# Autodesk Inventor assembly: Assembly1
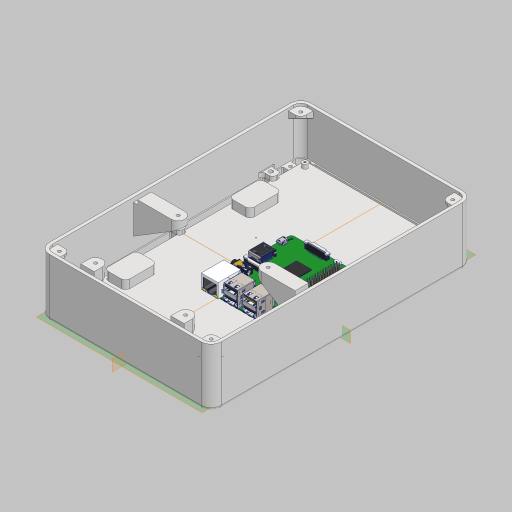
[picture p0: Inventor's stored thumbnail of the model, 512x512]
Saved by Autodesk Inventor 2024 (Build 280153000, 153)
## iProperties
Created: 2024-11-22
Part Number: Assembly1
Document SubType Name: Assembly
Designer: Stefano
Author: Stefano
## Documents named in this file (8)
- C:\Users\Stefano\Documents\Inventor\Provvedo\inventor-dro-case\wisecoco-10-version\Assembly1.iam
- C:\Users\Stefano\Documents\Inventor\Provvedo\inventor-dro-case\wisecoco-10-version\wisecoco-display.ipt
- C:\Users\Stefano\Documents\Inventor\Provvedo\inventor-dro-case\waveshare-10-version\front-bezel.ipt
- C:\Users\Stefano\Documents\Inventor\Provvedo\inventor-dro-case\wisecoco-10-version\display-retainer-tab.ipt
- C:\Users\Stefano\Documents\Inventor\Provvedo\inventor-dro-case\wisecoco-10-version\enclosure-body.ipt
- C:\Users\Stefano\Documents\Inventor\Provvedo\inventor-dro-case\wisecoco-10-version\Raspberry Pi 3 .ipt
- C:\Users\Stefano\Documents\Inventor\Provvedo\inventor-dro-case\wisecoco-10-version\STEP\back-cover.ipt
- C:\Users\Stefano\Documents\Inventor\Provvedo\inventor-dro-case\wisecoco-10-version\barrel-receptacle.ipt
## Components (7 placed, 7 different names)
1. wisecoco-display:1 — Flush:1, Flush:2, Mate:1, Mate:2, Mate:5, Mate:6, Mate:7
2. front-bezel:1 — Flush:1, Flush:2, Mate:3, Mate:4, Flush:3
3. display-retainer-tab:1 — Mate:1, Mate:2
4. enclosure-body:1 — Mate:3, Mate:4, Flush:3, Flush:4, Flush:5
5. Raspberry Pi 3 :1 — Mate:5, Mate:6, Mate:7
6. back-cover:1 — Flush:4, Flush:5, Mate:15, Mate:16
7. barrel-receptacle:1 — Mate:15, Mate:16
## Relationships (14: Mate 9, Flush 5)
- Flush:1: wisecoco-display:1 ↔ front-bezel:1
- Flush:2: wisecoco-display:1 ↔ front-bezel:1
- Mate:1: wisecoco-display:1 ↔ display-retainer-tab:1
- Mate:2: wisecoco-display:1 ↔ display-retainer-tab:1
- Mate:3: front-bezel:1 ↔ enclosure-body:1
- Mate:4: front-bezel:1 ↔ enclosure-body:1
- Flush:3: front-bezel:1 ↔ enclosure-body:1
- Mate:5: wisecoco-display:1 ↔ Raspberry Pi 3 :1
- Mate:6: wisecoco-display:1 ↔ Raspberry Pi 3 :1
- Mate:7: wisecoco-display:1 ↔ Raspberry Pi 3 :1
- Flush:4: enclosure-body:1 ↔ back-cover:1
- Flush:5: enclosure-body:1 ↔ back-cover:1
- Mate:15: back-cover:1 ↔ barrel-receptacle:1
- Mate:16: back-cover:1 ↔ barrel-receptacle:1
